# Autodesk Inventor assembly: Stock Dicoeasy Assembly-rebuild test
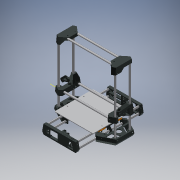
[picture p0: Inventor's stored thumbnail of the model, 180x180]
Saved by Autodesk Inventor 2017 (Build 210142000, 142)
## iProperties
Created: 2017-03-10
Part Number: Stock Dicoeasy Assembly-rebuild test
Document SubType Name: Assembly
Designer: gilef
Author: gilef
## Documents named in this file (17)
- C:\Users\gilef\Documents\Inventor\DiscoEasy200\Stock Dicoeasy Assembly-rebuild test.iam
- C:\Users\gilef\Documents\Inventor\DiscoEasy200\Original Plate Mount.ipt
- C:\Users\gilef\Documents\Inventor\DiscoEasy200\Original Rear Left Plate Mount.ipt
- C:\Users\gilef\Documents\Inventor\DiscoEasy200\Original Rear Right Plate Mount.ipt
- C:\Users\gilef\Documents\Inventor\DiscoEasy200\Converted LM8UU Linear Bearing.ipt
- C:\Users\gilef\Documents\Inventor\DiscoEasy200\Stock Build Plate.ipt
- C:\Users\gilef\Documents\Inventor\Content Center Files\R2017\en-US\AS 1427(07)\AS 1427 - M3 x 10(6) II.ipt
- C:\Users\gilef\Documents\Inventor\Content Center Files\R2017\en-US\ANSI B18.16.3M(2)\ANSI B18.16.3M - Property Class 5 and 10 - Metric M3 x 0.5 Metal Type.ipt
- C:\Users\gilef\Documents\Inventor\DiscoEasy200\Stock Front Plate.ipt
- C:\Users\gilef\Documents\Inventor\DiscoEasy200\Stock Back Plate.ipt
- C:\Users\gilef\Documents\Inventor\DiscoEasy200\Long Metal Rod.ipt
- C:\Users\gilef\Documents\Inventor\DiscoEasy200\Short Metal Rod.ipt
- C:\Users\gilef\Documents\Inventor\DiscoEasy200\Original Printer Base.ipt
- C:\Users\gilef\Documents\Inventor\DiscoEasy200\Stock Left Top.ipt
- C:\Users\gilef\Documents\Inventor\DiscoEasy200\Stock Top Right.ipt
- C:\Users\gilef\Documents\Inventor\DiscoEasy200\Stock X Axis Left (Extruder).ipt
- C:\Users\gilef\Documents\Inventor\DiscoEasy200\Stock X Axis Right.ipt
## Components (37 placed, 16 different names)
1. Original Plate Mount:1 — Flush:2, Mate:1, Flush:3, Mate:2, Mate:7, Mate:8, Mate:9, Mate:10, Mate:11, Insert:7, Angle:3, Insert:10, Angle:4
2. Original Rear Right Plate Mount:1 — Flush:2, Mate:1, Mate:3, Mate:4, Flush:4, Insert:9, Angle:1
3. Original Rear Left Plate Mount:1 — Flush:3, Mate:2, Mate:5, Mate:6, Flush:4, Insert:1, Insert:6, Angle:2
4. Converted LM8UU Linear Bearing:1 — Mate:7, Mate:8, Mate:15
5. Converted LM8UU Linear Bearing:2 — Mate:3, Mate:4, Mate:12
6. Converted LM8UU Linear Bearing:3 — Mate:9, Mate:10, Mate:14
7. Converted LM8UU Linear Bearing:4 — Mate:5, Mate:6, Mate:13
8. Stock Build Plate:1 — Insert:1, Mate:11, Insert:2, Insert:3, Insert:4, Insert:5
9. AS 1427 Z - Metric M3 x 10:1 — Insert:2
10. AS 1427 Z - Metric M3 x 10:2 — Insert:3
11. AS 1427 Z - Metric M3 x 10:3 — Insert:4
12. AS 1427 Z - Metric M3 x 10:4 — Insert:5
13. Prevailing Torque Type Hex Nut - Steel Metric Property Class 5 and 10 - Metric M3 x 0.5 Metal Type:1 — Insert:10, Angle:4
14. Prevailing Torque Type Hex Nut - Steel Metric Property Class 5 and 10 - Metric M3 x 0.5 Metal Type:2 — Insert:9, Angle:1
15. Prevailing Torque Type Hex Nut - Steel Metric Property Class 5 and 10 - Metric M3 x 0.5 Metal Type:3 — Insert:7, Angle:3
16. Prevailing Torque Type Hex Nut - Steel Metric Property Class 5 and 10 - Metric M3 x 0.5 Metal Type:4 — Insert:6, Angle:2
17. Stock Front Plate:1 — Mate:14, Mate:15, Mate:18, Mate:21, Mate:22, Flush:5
18. Stock Back Plate:1 — Mate:12, Mate:13, Mate:16, Mate:17, Mate:19, Mate:20, Mate:23, Mate:24
19. Long Metal Rod:1 — Mate:16, Mate:17, Mate:18, Mate:25
20. Long Metal Rod:2 — Mate:19, Mate:20
21. Long Metal Rod:3 — Mate:21, Mate:22
22. Long Metal Rod:4 — Mate:23, Mate:24, Mate:26
23. Short Metal Rod:1 — Mate:27, Mate:28, Mate:29
24. Original Printer Base:1 — Flush:6, Mate:26, Mate:28, Mate:29, Mate:32, Mate:33, Mate:36, Mate:37
25. Original Printer Base:2 — Mate:25, Flush:5, Flush:6, Mate:27, Mate:30, Mate:31, Mate:34, Mate:35
26. Long Metal Rod:5 — Mate:30, Mate:35, Mate:42, Mate:50
27. Long Metal Rod:6 — Mate:31, Mate:34, Mate:41, Mate:43, Mate:51
28. Long Metal Rod:7 — Mate:32, Mate:36, Mate:38, Mate:40, Mate:49
29. Long Metal Rod:8 — Mate:33, Mate:37, Mate:39, Mate:48
30. Stock Left Top:1 — Mate:41, Mate:42, Mate:43, Mate:45, Mate:47
31. Stock Top Right:1 — Mate:38, Mate:39, Mate:40, Mate:44, Mate:46
32. Short Metal Rod:2 — Mate:44, Mate:45
33. Short Metal Rod:3 — Mate:46, Mate:47
34. Stock X Axis Left (Extruder):1 — Mate:48, Mate:49, Mate:53, Insert:11, Insert:12
35. Stock X Axis Right:1 — Mate:50, Mate:51
36. Short Metal Rod:4 — Insert:11
37. Short Metal Rod:5 — Insert:12
## Relationships (72: Mate 52, Insert 11, Flush 5, Angle 4)
- Flush:2: Original Plate Mount:1 ↔ Original Rear Right Plate Mount:1
- Mate:1: Original Plate Mount:1 ↔ Original Rear Right Plate Mount:1
- Flush:3: Original Plate Mount:1 ↔ Original Rear Left Plate Mount:1
- Mate:2: Original Plate Mount:1 ↔ Original Rear Left Plate Mount:1
- Mate:3: Original Rear Right Plate Mount:1 ↔ Converted LM8UU Linear Bearing:2
- Mate:4: Original Rear Right Plate Mount:1 ↔ Converted LM8UU Linear Bearing:2
- Mate:5: Original Rear Left Plate Mount:1 ↔ Converted LM8UU Linear Bearing:4
- Mate:6: Original Rear Left Plate Mount:1 ↔ Converted LM8UU Linear Bearing:4
- Mate:7: Original Plate Mount:1 ↔ Converted LM8UU Linear Bearing:1
- Mate:8: Original Plate Mount:1 ↔ Converted LM8UU Linear Bearing:1
- Mate:9: Original Plate Mount:1 ↔ Converted LM8UU Linear Bearing:3
- Mate:10: Original Plate Mount:1 ↔ Converted LM8UU Linear Bearing:3
- Flush:4: Original Rear Right Plate Mount:1 ↔ Original Rear Left Plate Mount:1
- Insert:1: Original Rear Left Plate Mount:1 ↔ Stock Build Plate:1
- Mate:11: Original Plate Mount:1 ↔ Stock Build Plate:1
- Insert:2: Stock Build Plate:1 ↔ AS 1427 Z - Metric M3 x 10:1
- Insert:3: Stock Build Plate:1 ↔ AS 1427 Z - Metric M3 x 10:2
- Insert:4: Stock Build Plate:1 ↔ AS 1427 Z - Metric M3 x 10:3
- Insert:5: Stock Build Plate:1 ↔ AS 1427 Z - Metric M3 x 10:4
- Insert:6: Original Rear Left Plate Mount:1 ↔ Prevailing Torque Type Hex Nut - Steel Metric Property Class 5 and 10 - Metric M3 x 0.5 Metal Type:4
- Insert:7: Original Plate Mount:1 ↔ Prevailing Torque Type Hex Nut - Steel Metric Property Class 5 and 10 - Metric M3 x 0.5 Metal Type:3
- Insert:9: Original Rear Right Plate Mount:1 ↔ Prevailing Torque Type Hex Nut - Steel Metric Property Class 5 and 10 - Metric M3 x 0.5 Metal Type:2
- Angle:1 (0 deg): Original Rear Right Plate Mount:1 ↔ Prevailing Torque Type Hex Nut - Steel Metric Property Class 5 and 10 - Metric M3 x 0.5 Metal Type:2
- Angle:2 (0 deg): Original Rear Left Plate Mount:1 ↔ Prevailing Torque Type Hex Nut - Steel Metric Property Class 5 and 10 - Metric M3 x 0.5 Metal Type:4
- Angle:3 (0 deg): Original Plate Mount:1 ↔ Prevailing Torque Type Hex Nut - Steel Metric Property Class 5 and 10 - Metric M3 x 0.5 Metal Type:3
- Insert:10: Original Plate Mount:1 ↔ Prevailing Torque Type Hex Nut - Steel Metric Property Class 5 and 10 - Metric M3 x 0.5 Metal Type:1
- Angle:4 (0 deg): Original Plate Mount:1 ↔ Prevailing Torque Type Hex Nut - Steel Metric Property Class 5 and 10 - Metric M3 x 0.5 Metal Type:1
- Mate:12: Converted LM8UU Linear Bearing:2 ↔ Stock Back Plate:1
- Mate:13: Converted LM8UU Linear Bearing:4 ↔ Stock Back Plate:1
- Mate:14: Converted LM8UU Linear Bearing:3 ↔ Stock Front Plate:1
- Mate:15: Converted LM8UU Linear Bearing:1 ↔ Stock Front Plate:1
- Mate:16: Stock Back Plate:1 ↔ Long Metal Rod:1
- Mate:17: Stock Back Plate:1 ↔ Long Metal Rod:1
- Mate:18: Stock Front Plate:1 ↔ Long Metal Rod:1
- Mate:19: Stock Back Plate:1 ↔ Long Metal Rod:2
- Mate:20: Stock Back Plate:1 ↔ Long Metal Rod:2
- Mate:21: Stock Front Plate:1 ↔ Long Metal Rod:3
- Mate:22: Stock Front Plate:1 ↔ Long Metal Rod:3
- Mate:23: Stock Back Plate:1 ↔ Long Metal Rod:4
- Mate:24: Stock Back Plate:1 ↔ Long Metal Rod:4
- Mate:25: Long Metal Rod:1 ↔ Original Printer Base:2
- Flush:5: Stock Front Plate:1 ↔ Original Printer Base:2
- Flush:6: Original Printer Base:1 ↔ Original Printer Base:2
- Mate:26: Long Metal Rod:4 ↔ Original Printer Base:1
- Mate:27: Short Metal Rod:1 ↔ Original Printer Base:2
- Mate:28: Short Metal Rod:1 ↔ Original Printer Base:1
- Mate:29: Short Metal Rod:1 ↔ Original Printer Base:1
- Mate:30: Original Printer Base:2 ↔ Long Metal Rod:5
- Mate:31: Original Printer Base:2 ↔ Long Metal Rod:6
- Mate:32: Original Printer Base:1 ↔ Long Metal Rod:7
- Mate:33: Original Printer Base:1 ↔ Long Metal Rod:8
- Mate:34: Original Printer Base:2 ↔ Long Metal Rod:6
- Mate:35: Original Printer Base:2 ↔ Long Metal Rod:5
- Mate:36: Original Printer Base:1 ↔ Long Metal Rod:7
- Mate:37: Original Printer Base:1 ↔ Long Metal Rod:8
- Mate:38: Long Metal Rod:7 ↔ Stock Top Right:1
- Mate:39: Long Metal Rod:8 ↔ Stock Top Right:1
- Mate:40: Long Metal Rod:7 ↔ Stock Top Right:1
- Mate:41: Long Metal Rod:6 ↔ Stock Left Top:1
- Mate:42: Long Metal Rod:5 ↔ Stock Left Top:1
- Mate:43: Long Metal Rod:6 ↔ Stock Left Top:1
- Mate:44: Stock Top Right:1 ↔ Short Metal Rod:2
- Mate:45: Stock Left Top:1 ↔ Short Metal Rod:2
- Mate:46: Stock Top Right:1 ↔ Short Metal Rod:3
- Mate:47: Stock Left Top:1 ↔ Short Metal Rod:3
- Mate:48: Long Metal Rod:8 ↔ Stock X Axis Left (Extruder):1
- Mate:49: Long Metal Rod:7 ↔ Stock X Axis Left (Extruder):1
- Mate:50: Long Metal Rod:5 ↔ Stock X Axis Right:1
- Mate:51: Long Metal Rod:6 ↔ Stock X Axis Right:1
- Mate:53: Stock X Axis Left (Extruder):1
- Insert:11: Stock X Axis Left (Extruder):1 ↔ Short Metal Rod:4
- Insert:12: Stock X Axis Left (Extruder):1 ↔ Short Metal Rod:5
